# Autodesk Inventor assembly: PeltierController
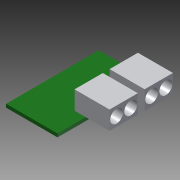
[picture p0: Inventor's stored thumbnail of the model, 180x180]
Saved by Autodesk Inventor 2014 (Build 180170000, 170)
## iProperties
Created: 2015-04-19
Part Number: PeltierController
Document SubType Name: Assembly
Designer: Owner
Author: Owner
## Documents named in this file (3)
- C:\Users\Owner\Documents\APC\FrontEnd\IAM\Common\PeltierController.iam
- C:\Users\Owner\Documents\APC\FrontEnd\IAM\Common\PeltierControllerBoard.ipt
- C:\Users\Owner\Documents\APC\FrontEnd\IAM\Common\TE_2Pin.ipt
## Components (3 placed, 2 different names)
1. PeltierControllerBoard:1 — Mate:1, Mate:2, Flush:1, Flush:2, Flush:3, Flush:4
2. TE_2Pin:1 — Mate:1, Flush:2, Flush:3
3. TE_2Pin:2 — Mate:2, Flush:1, Flush:4
## Relationships (6: Flush 4, Mate 2)
- Mate:1: PeltierControllerBoard:1 ↔ TE_2Pin:1
- Mate:2: PeltierControllerBoard:1 ↔ TE_2Pin:2
- Flush:1 (19.8679 mm): PeltierControllerBoard:1 ↔ TE_2Pin:2
- Flush:2 (-19.8679 mm): PeltierControllerBoard:1 ↔ TE_2Pin:1
- Flush:3 (0.4953 mm): PeltierControllerBoard:1 ↔ TE_2Pin:1
- Flush:4 (17.8206 mm): PeltierControllerBoard:1 ↔ TE_2Pin:2
